# Autodesk Inventor assembly: アームマウント
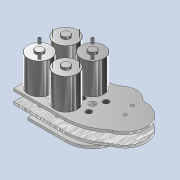
[picture p0: Inventor's stored thumbnail of the model, 180x180]
Saved by Autodesk Inventor 2020.4 (Build 244396000, 396)
## iProperties
Created: 2021-04-23
Part Number: アームマウント
Document SubType Name: Assembly
Designer: happy
Author: happy
## Documents named in this file (9)
- C:\Users\happy\OneDrive\ドキュメント\賢一ファイル\SRDC\試作10-2\excel\アームマウント.iam
- C:\Users\happy\OneDrive\ドキュメント\賢一ファイル\SRDC\試作10-2\アームギア\外側フレーム.ipt
- C:\Users\happy\OneDrive\ドキュメント\賢一ファイル\SRDC\試作10-2\アームギア\最終段小ギア軸受け.ipt
- C:\Users\happy\OneDrive\ドキュメント\賢一ファイル\SRDC\試作10-2\アームギア\中間フレーム.ipt
- C:\Users\happy\OneDrive\ドキュメント\賢一ファイル\SRDC\試作10-2\モータ\アームモータマウント.ipt
- C:\Users\happy\OneDrive\ドキュメント\賢一ファイル\SRDC\試作10-2\モータ\アームモータマウント軸受けパーツ.ipt
- C:\Users\happy\OneDrive\ドキュメント\賢一ファイル\SRDC\試作10-2\モータ\RS-380.ipt
- C:\Users\happy\OneDrive\ドキュメント\賢一ファイル\SRDC\試作10-2\ねじ\m2.6 6mm キャップボルト.ipt
- C:\Users\happy\OneDrive\ドキュメント\賢一ファイル\SRDC\試作10-2\ねじ\m3皿ネジ6.ipt
## Components (20 placed, 8 different names)
1. 外側フレーム:1 — メイト:3, メイト:4, メイト:6
2. 最終段小ギア軸受け:1 — 挿入:3, 挿入:4
3. 中間フレーム:1 — メイト:1, メイト:2, メイト:3, メイト:4, メイト:5, メイト:6
4. アームモータマウント:1 — 挿入:1, 挿入:2, 挿入:3, 挿入:4, メイト:1, メイト:2, メイト:5, 挿入:5, 挿入:6, 挿入:7, 挿入:8, 挿入:9, 挿入:10, 挿入:11, 挿入:12, 挿入:13, 挿入:14, 挿入:15, 挿入:16, 挿入:17, 挿入:18, 挿入:19, 挿入:20, 挿入:21, 挿入:22, 挿入:23
5. アームモータマウント軸受けパーツ:1 — 挿入:1, 挿入:2
6. RS-380:1 — 挿入:5, 挿入:6
7. RS-380:2 — 挿入:11, 挿入:12
8. RS-380:3 — 挿入:7, 挿入:8
9. RS-380:4 — 挿入:9, 挿入:10
10. m2.6 6mm キャップボルト:1 — 挿入:13
11. m2.6 6mm キャップボルト:2 — 挿入:14
12. m2.6 6mm キャップボルト:3 — 挿入:15
13. m2.6 6mm キャップボルト:4 — 挿入:16
14. m2.6 6mm キャップボルト:5 — 挿入:17
15. m2.6 6mm キャップボルト:6 — 挿入:18
16. m2.6 6mm キャップボルト:7 — 挿入:19
17. m2.6 6mm キャップボルト:8 — 挿入:20
18. m3皿ネジ6:1 — 挿入:21
19. m3皿ネジ6:2 — 挿入:22
20. m3皿ネジ6:3 — 挿入:23
## Relationships (29: Insert 23, Mate 6)
- 挿入:1 [Insert]: アームモータマウント:1 ↔ アームモータマウント軸受けパーツ:1
- 挿入:2 [Insert]: アームモータマウント:1 ↔ アームモータマウント軸受けパーツ:1
- 挿入:3 [Insert]: 最終段小ギア軸受け:1 ↔ アームモータマウント:1
- 挿入:4 [Insert]: 最終段小ギア軸受け:1 ↔ アームモータマウント:1
- メイト:1 [Mate]: 中間フレーム:1 ↔ アームモータマウント:1
- メイト:2 [Mate]: 中間フレーム:1 ↔ アームモータマウント:1
- メイト:3 [Mate]: 外側フレーム:1 ↔ 中間フレーム:1
- メイト:4 [Mate]: 外側フレーム:1 ↔ 中間フレーム:1
- メイト:5 [Mate] (11 mm): 中間フレーム:1 ↔ アームモータマウント:1
- メイト:6 [Mate] (5 mm): 外側フレーム:1 ↔ 中間フレーム:1
- 挿入:5 [Insert]: アームモータマウント:1 ↔ RS-380:1
- 挿入:6 [Insert]: アームモータマウント:1 ↔ RS-380:1
- 挿入:7 [Insert]: アームモータマウント:1 ↔ RS-380:3
- 挿入:8 [Insert]: アームモータマウント:1 ↔ RS-380:3
- 挿入:9 [Insert]: アームモータマウント:1 ↔ RS-380:4
- 挿入:10 [Insert]: アームモータマウント:1 ↔ RS-380:4
- 挿入:11 [Insert]: アームモータマウント:1 ↔ RS-380:2
- 挿入:12 [Insert]: アームモータマウント:1 ↔ RS-380:2
- 挿入:13 [Insert]: アームモータマウント:1 ↔ m2.6 6mm キャップボルト:1
- 挿入:14 [Insert]: アームモータマウント:1 ↔ m2.6 6mm キャップボルト:2
- 挿入:15 [Insert]: アームモータマウント:1 ↔ m2.6 6mm キャップボルト:3
- 挿入:16 [Insert]: アームモータマウント:1 ↔ m2.6 6mm キャップボルト:4
- 挿入:17 [Insert]: アームモータマウント:1 ↔ m2.6 6mm キャップボルト:5
- 挿入:18 [Insert]: アームモータマウント:1 ↔ m2.6 6mm キャップボルト:6
- 挿入:19 [Insert]: アームモータマウント:1 ↔ m2.6 6mm キャップボルト:7
- 挿入:20 [Insert]: アームモータマウント:1 ↔ m2.6 6mm キャップボルト:8
- 挿入:21 [Insert]: アームモータマウント:1 ↔ m3皿ネジ6:1
- 挿入:22 [Insert]: アームモータマウント:1 ↔ m3皿ネジ6:2
- 挿入:23 [Insert]: アームモータマウント:1 ↔ m3皿ネジ6:3
